# Autodesk Inventor assembly: Hoja Oculta
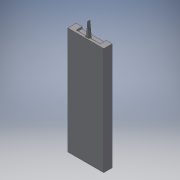
[picture p0: Inventor's stored thumbnail of the model, 180x180]
Saved by Autodesk Inventor 2017 (Build 210142000, 142)
## iProperties
Created: 2017-01-19
Part Number: Hoja Oculta
Document SubType Name: Assembly
Designer: A. Matías Quezada
Author: A. Matías Quezada
## Documents named in this file (6)
- D:\repos\3D\Hoja Oculta\Prototipo\Hoja Oculta.iam
- D:\repos\3D\Hoja Oculta\Prototipo\Base.ipt
- D:\repos\3D\Hoja Oculta\Prototipo\Hoja.ipt
- D:\repos\3D\Hoja Oculta\Prototipo\Tirador.ipt
- D:\repos\3D\Hoja Oculta\Prototipo\Deslizador.ipt
- D:\repos\3D\Hoja Oculta\Prototipo\Parametros.ipt
## Components (5 placed, 4 different names)
1. Base:1 — Movimiento Hoja, Limites Hoja, Limites Tirador 2, Limites Tirador 1, Slider:4, Slider:5, Slider:6
2. Hoja:1 — Movimiento Hoja, Limites Hoja, Mate:7, Mate:8
3. Tirador:1 — Limites Tirador 1, Mate:6, Slider:6, Mate:8
4. Tirador:2 — Limites Tirador 2, Mate:5, Slider:5, Mate:7
5. Deslizador:1 — Slider:4, Mate:5, Mate:6
## Relationships (11: Mate 7, TranslationJoint 4)
- Movimiento Hoja [TranslationJoint] (1 mm): Base:1 ↔ Hoja:1
- Limites Hoja [Mate]: Base:1 ↔ Hoja:1
- Limites Tirador 2 [Mate]: Base:1 ↔ Tirador:2
- Limites Tirador 1 [Mate]: Base:1 ↔ Tirador:1
- Slider:4 [TranslationJoint]: Base:1 ↔ Deslizador:1
- Mate:5: Tirador:2 ↔ Deslizador:1
- Mate:6: Tirador:1 ↔ Deslizador:1
- Slider:5 [TranslationJoint]: Base:1 ↔ Tirador:2
- Slider:6 [TranslationJoint]: Base:1 ↔ Tirador:1
- Mate:7: Hoja:1 ↔ Tirador:2
- Mate:8: Hoja:1 ↔ Tirador:1
## Named parameters: movimiento_deslizador = 41 mm, movimiento_hoja = 133 mm
